# Autodesk Inventor assembly: giant-midi-keyboard
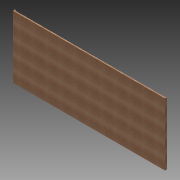
[picture p0: Inventor's stored thumbnail of the model, 180x180]
Saved by Autodesk Inventor 2014 SP1 (Build 180222100, 222)
## iProperties
Created: 2015-03-28
Part Number: giant-midi-keyboard
Document SubType Name: Assembly
Designer: tuleu
Author: tuleu
## Documents named in this file (12)
- C:\Users\tuleu\Documents\giant-midi-keyboard\cad\mechanics\giant-midi-keyboard.iam
- C:\Users\tuleu\Documents\giant-midi-keyboard\cad\mechanics\Base.ipt
- C:\Users\tuleu\Documents\giant-midi-keyboard\cad\mechanics\Do.ipt
- C:\Users\tuleu\Documents\giant-midi-keyboard\cad\mechanics\Captor.ipt
- C:\Users\tuleu\Documents\giant-midi-keyboard\cad\mechanics\Re.ipt
- C:\Users\tuleu\Documents\giant-midi-keyboard\cad\mechanics\Mi.ipt
- C:\Users\tuleu\Documents\giant-midi-keyboard\cad\mechanics\Fa.ipt
- C:\Users\tuleu\Documents\giant-midi-keyboard\cad\mechanics\Sol.ipt
- C:\Users\tuleu\Documents\giant-midi-keyboard\cad\mechanics\La.ipt
- C:\Users\tuleu\Documents\giant-midi-keyboard\cad\mechanics\Si.ipt
- C:\Users\tuleu\Documents\giant-midi-keyboard\cad\mechanics\Do_Plain.ipt
- C:\Users\tuleu\Documents\giant-midi-keyboard\cad\mechanics\Feinte.ipt
## Components (51 placed, 11 different names)
1. Base:1 — Mate:6, Flush:1, Mate:7, Mate:8, Mate:9, Mate:10, Mate:11, Mate:12, Mate:13, Mate:14, Mate:15, Mate:16, Mate:17, Flush:11, Mate:18, Flush:22, Mate:19, Mate:20, Flush:23, Mate:22, Flush:24, Mate:24, Flush:25, Mate:26, Flush:26, Mate:28, Flush:27, Mate:30, Flush:28, Mate:32, Flush:29, Mate:34, Flush:30, Mate:36, Flush:31, Mate:38, Flush:32, Mate:40, Flush:33, Mate:42, Flush:34, Mate:44, Flush:35, Mate:46, Mate:47, Flush:36, Mate:58, Mate:59, Mate:60, Mate:61, Mate:62, Mate:63, Mate:64, Mate:65, Mate:66, Mate:67, Flush:46
2. Do:1 — Mate:18, Flush:22, Mate:19, Mate:21, Mate:48, Mate:68
3. Do:2 — Mate:32, Mate:33, Flush:29, Mate:35, Mate:53
4. Captor:16 — Mate:8, Flush:2, Flush:11, Mate:48
5. Captor:17 — Mate:9, Flush:2, Flush:3, Mate:49
6. Captor:18 — Mate:10, Flush:3, Flush:4, Mate:50
7. Captor:19 — Mate:11, Flush:4, Flush:5, Mate:51
8. Captor:20 — Mate:12, Flush:5, Flush:6, Mate:52
9. Captor:21 — Mate:13, Flush:6, Flush:7, Mate:53
10. Captor:22 — Mate:14, Flush:7, Flush:8, Mate:54
11. Captor:23 — Mate:15, Flush:8, Flush:9, Mate:55
12. Captor:24 — Mate:16, Flush:9, Flush:10, Mate:56
13. Captor:25 — Mate:17, Flush:10, Mate:57
14. Re:1 — Mate:20, Flush:23, Mate:21, Mate:23, Mate:49, Mate:69
15. Re:2 — Mate:34, Mate:35, Flush:30, Mate:37, Mate:54, Mate:73, Mate:74
16. Mi:1 — Mate:22, Flush:24, Mate:23, Mate:25
17. Mi:2 — Mate:36, Mate:37, Flush:31, Mate:39
18. Fa:1 — Mate:24, Flush:25, Mate:25, Mate:27, Mate:50, Mate:70
19. Fa:2 — Mate:38, Mate:39, Flush:32, Mate:41, Mate:55
20. Sol:1 — Mate:26, Mate:27, Flush:26, Mate:29, Mate:51
21. Sol:2 — Mate:40, Mate:41, Flush:33, Mate:43, Mate:56, Mate:75
22. La:1 — Mate:28, Mate:29, Flush:27, Mate:31, Mate:52, Mate:71
23. La:2 — Mate:42, Mate:43, Flush:34, Mate:45, Mate:57, Mate:76
24. Si:1 — Mate:30, Mate:31, Flush:28, Mate:33, Mate:72
25. Si:2 — Mate:44, Mate:45, Flush:35, Mate:77
26. Do_Plain:1 — Mate:46, Mate:47, Flush:36
27. Feinte:1 — Mate:58, Flush:45, Mate:69
28. Feinte:2 — Mate:59, Flush:37, Flush:45, Flush:46, Mate:68
29. Feinte:3 — Mate:60, Flush:37, Flush:38, Mate:70
30. Feinte:4 — Mate:61, Flush:38, Flush:39, Mate:71
31. Feinte:5 — Mate:62, Flush:39, Flush:40, Mate:72
32. Feinte:6 — Mate:63, Flush:40, Flush:41, Mate:73
33. Feinte:7 — Mate:64, Flush:41, Flush:42, Mate:74
34. Feinte:8 — Mate:65, Flush:42, Flush:43, Mate:75
35. Feinte:9 — Mate:66, Flush:43, Flush:44, Mate:76
36. Feinte:10 — Mate:67, Flush:44, Mate:77
37. Captor:1 — Mate:6, Flush:1, Mate:7
38. Captor:2
39. Captor:3
40. Captor:4
41. Captor:5
42. Captor:6
43. Captor:7
44. Captor:8
45. Captor:9
46. Captor:10
47. Captor:11
48. Captor:12
49. Captor:13
50. Captor:14
51. Captor:15
## Component patterns: (15 elements, first: Captor:1)
## Relationships (108: Mate 72, Flush 36)
- Mate:6: Base:1 ↔ Captor:1
- Flush:1 (50 mm): Base:1 ↔ Captor:1
- Mate:7 (50 mm): Base:1 ↔ Captor:1
- Mate:8: Base:1 ↔ Captor:16
- Mate:9: Base:1 ↔ Captor:17
- Mate:10: Base:1 ↔ Captor:18
- Mate:11: Base:1 ↔ Captor:19
- Mate:12: Base:1 ↔ Captor:20
- Mate:13: Base:1 ↔ Captor:21
- Mate:14: Base:1 ↔ Captor:22
- Mate:15: Base:1 ↔ Captor:23
- Mate:16: Base:1 ↔ Captor:24
- Mate:17: Base:1 ↔ Captor:25
- Flush:2: Captor:16 ↔ Captor:17
- Flush:3: Captor:17 ↔ Captor:18
- Flush:4: Captor:18 ↔ Captor:19
- Flush:5: Captor:19 ↔ Captor:20
- Flush:6: Captor:20 ↔ Captor:21
- Flush:7: Captor:21 ↔ Captor:22
- Flush:8: Captor:22 ↔ Captor:23
- Flush:9: Captor:23 ↔ Captor:24
- Flush:10: Captor:24 ↔ Captor:25
- Flush:11 (450 mm): Base:1 ↔ Captor:16
- Mate:18: Base:1 ↔ Do:1
- Flush:22: Base:1 ↔ Do:1
- Mate:19: Base:1 ↔ Do:1
- Mate:20: Base:1 ↔ Re:1
- Flush:23: Base:1 ↔ Re:1
- Mate:21 (5 mm): Do:1 ↔ Re:1
- Mate:22: Base:1 ↔ Mi:1
- Flush:24: Base:1 ↔ Mi:1
- Mate:23 (5 mm): Re:1 ↔ Mi:1
- Mate:24: Base:1 ↔ Fa:1
- Flush:25: Base:1 ↔ Fa:1
- Mate:25 (5 mm): Mi:1 ↔ Fa:1
- Mate:26: Base:1 ↔ Sol:1
- Mate:27 (5 mm): Fa:1 ↔ Sol:1
- Flush:26: Base:1 ↔ Sol:1
- Mate:28: Base:1 ↔ La:1
- Mate:29 (5 mm): Sol:1 ↔ La:1
- Flush:27: Base:1 ↔ La:1
- Mate:30: Base:1 ↔ Si:1
- Mate:31 (5 mm): La:1 ↔ Si:1
- Flush:28: Base:1 ↔ Si:1
- Mate:32: Base:1 ↔ Do:2
- Mate:33 (5 mm): Do:2 ↔ Si:1
- Flush:29: Base:1 ↔ Do:2
- Mate:34: Base:1 ↔ Re:2
- Mate:35 (5 mm): Do:2 ↔ Re:2
- Flush:30: Base:1 ↔ Re:2
- Mate:36: Base:1 ↔ Mi:2
- Mate:37 (5 mm): Re:2 ↔ Mi:2
- Flush:31: Base:1 ↔ Mi:2
- Mate:38: Base:1 ↔ Fa:2
- Mate:39 (5 mm): Mi:2 ↔ Fa:2
- Flush:32: Base:1 ↔ Fa:2
- Mate:40: Base:1 ↔ Sol:2
- Mate:41 (5 mm): Fa:2 ↔ Sol:2
- Flush:33: Base:1 ↔ Sol:2
- Mate:42: Base:1 ↔ La:2
- Mate:43 (5 mm): Sol:2 ↔ La:2
- Flush:34: Base:1 ↔ La:2
- Mate:44: Base:1 ↔ Si:2
- Mate:45 (5 mm): La:2 ↔ Si:2
- Flush:35: Base:1 ↔ Si:2
- Mate:46: Base:1 ↔ Do_Plain:1
- Mate:47: Base:1 ↔ Do_Plain:1
- Flush:36: Base:1 ↔ Do_Plain:1
- Mate:48 (17.5 mm): Do:1 ↔ Captor:16
- Mate:49 (17.5 mm): Captor:17 ↔ Re:1
- Mate:50 (17.5 mm): Captor:18 ↔ Fa:1
- Mate:51 (17.5 mm): Captor:19 ↔ Sol:1
- Mate:52 (17.5 mm): Captor:20 ↔ La:1
- Mate:53 (17.5 mm): Do:2 ↔ Captor:21
- Mate:54 (17.5 mm): Captor:22 ↔ Re:2
- Mate:55 (17.5 mm): Captor:23 ↔ Fa:2
- Mate:56 (17.5 mm): Captor:24 ↔ Sol:2
- Mate:57 (17.5 mm): Captor:25 ↔ La:2
- Mate:58: Base:1 ↔ Feinte:1
- Mate:59: Base:1 ↔ Feinte:2
- Mate:60: Base:1 ↔ Feinte:3
- Mate:61: Base:1 ↔ Feinte:4
- Mate:62: Base:1 ↔ Feinte:5
- Mate:63: Base:1 ↔ Feinte:6
- Mate:64: Base:1 ↔ Feinte:7
- Mate:65: Base:1 ↔ Feinte:8
- Mate:66: Base:1 ↔ Feinte:9
- Mate:67: Base:1 ↔ Feinte:10
- Flush:37: Feinte:2 ↔ Feinte:3
- Flush:38: Feinte:3 ↔ Feinte:4
- Flush:39: Feinte:4 ↔ Feinte:5
- Flush:40: Feinte:5 ↔ Feinte:6
- Flush:41: Feinte:6 ↔ Feinte:7
- Flush:42: Feinte:7 ↔ Feinte:8
- Flush:43: Feinte:8 ↔ Feinte:9
- Flush:44: Feinte:9 ↔ Feinte:10
- Flush:45: Feinte:1 ↔ Feinte:2
- Flush:46 (405 mm): Base:1 ↔ Feinte:2
- Mate:68 (5 mm): Do:1 ↔ Feinte:2
- Mate:69 (5 mm): Re:1 ↔ Feinte:1
- Mate:70 (5 mm): Fa:1 ↔ Feinte:3
- Mate:71 (5 mm): La:1 ↔ Feinte:4
- Mate:72 (5 mm): Si:1 ↔ Feinte:5
- Mate:73 (5 mm): Re:2 ↔ Feinte:6
- Mate:74 (5 mm): Re:2 ↔ Feinte:7
- Mate:75 (5 mm): Sol:2 ↔ Feinte:8
- Mate:76 (5 mm): La:2 ↔ Feinte:9
- Mate:77 (5 mm): Si:2 ↔ Feinte:10
